# Autodesk Inventor assembly: base
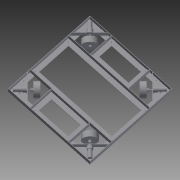
[picture p0: Inventor's stored thumbnail of the model, 180x180]
Saved by Autodesk Inventor 2015 (Build 190159000, 159)
## iProperties
Created: 2017-09-26
Part Number: base
Document SubType Name: Assembly
Designer: Anshul
Author: Anshul
## Documents named in this file (9)
- E:\robocon\throwing bot\base.iam
- E:\robocon\throwing bot\body_outer_L.ipt
- E:\robocon\throwing bot\body_inner_L_clamp.ipt
- E:\robocon\throwing bot\offcenter_L_clamp.ipt
- E:\robocon\throwing bot\offcentered_shaft_dc_and_encoder.ipt
- E:\robocon\throwing bot\omni_wheel.ipt
- E:\robocon\throwing bot\body_inner_center_bar.ipt
- E:\robocon\throwing bot\body_inner_L_support.ipt
- E:\robocon\throwing bot\body_inner_L_support(2).ipt
## Components (26 placed, 8 different names)
1. body_outer_L:1 — Mate:1, Flush:1, Mate:2, Flush:2, Mate:6, Mate:7, Mate:8, Mate:50, Mate:52
2. body_outer_L:2 — Mate:1, Flush:1, Mate:4, Mate:5, Mate:18, Mate:19, Mate:55, Mate:57, Mate:64, Mate:66
3. body_outer_L:3 — Mate:2, Flush:2, Mate:3, Flush:3, Mate:9, Mate:10, Mate:20, Mate:22, Mate:58, Mate:60, Mate:61, Mate:63
4. body_outer_L:4 — Mate:3, Mate:4, Flush:3, Mate:17, Mate:21, Mate:49, Mate:51, Mate:53, Mate:54
5. body_inner_L_clamp:1 — Mate:5, Mate:6, Mate:7, Mate:32, Mate:33, Mate:34
6. body_inner_L_clamp:2 — Mate:17, Mate:18, Mate:19, Mate:35, Mate:36, Mate:37
7. body_inner_L_clamp:3 — Mate:20, Mate:21, Mate:22, Mate:38, Mate:39, Mate:40
8. body_inner_L_clamp:4 — Mate:8, Mate:9, Mate:10, Mate:11, Mate:12, Mate:13
9. offcenter_L_clamp:1 — Mate:11, Mate:12, Mate:13, Mate:14, Mate:15, Mate:16
10. offcentered_shaft_dc_and_encoder:1 — Mate:14, Mate:15, Mate:16, Mate:45, Mate:48
11. offcenter_L_clamp:2 — Mate:35, Mate:36, Mate:37
12. offcentered_shaft_dc_and_encoder:2 — Mate:43, Mate:44
13. offcenter_L_clamp:3 — Mate:38, Mate:39, Mate:40
14. offcentered_shaft_dc_and_encoder:3 — Mate:46, Mate:47
15. offcenter_L_clamp:4 — Mate:32, Mate:33, Mate:34
16. offcentered_shaft_dc_and_encoder:4 — Mate:41, Mate:42
17. omni_wheel:1 — Mate:41, Mate:42
18. omni_wheel:2 — Mate:43, Mate:44
19. omni_wheel:3 — Mate:45, Mate:48
20. omni_wheel:4 — Mate:46, Mate:47
21. body_inner_center_bar:1 — Mate:49, Mate:50, Mate:54, Mate:59, Mate:62
22. body_inner_center_bar:2 — Mate:51, Mate:52, Mate:53, Mate:56, Mate:65
23. body_inner_L_support:1 — Mate:55, Mate:56, Mate:57
24. body_inner_L_support:2 — Mate:58, Mate:59, Mate:60
25. body_inner_L_support(2):1 — Mate:64, Mate:65, Mate:66
26. body_inner_L_support(2):2 — Mate:61, Mate:62, Mate:63
## Relationships (69: Mate 66, Flush 3)
- Mate:1: body_outer_L:1 ↔ body_outer_L:2
- Flush:1: body_outer_L:1 ↔ body_outer_L:2
- Mate:2: body_outer_L:1 ↔ body_outer_L:3
- Flush:2: body_outer_L:1 ↔ body_outer_L:3
- Mate:3: body_outer_L:3 ↔ body_outer_L:4
- Mate:4: body_outer_L:2 ↔ body_outer_L:4
- Flush:3: body_outer_L:3 ↔ body_outer_L:4
- Mate:5: body_outer_L:2 ↔ body_inner_L_clamp:1
- Mate:6: body_outer_L:1 ↔ body_inner_L_clamp:1
- Mate:7: body_outer_L:1 ↔ body_inner_L_clamp:1
- Mate:8: body_outer_L:1 ↔ body_inner_L_clamp:4
- Mate:9: body_outer_L:3 ↔ body_inner_L_clamp:4
- Mate:10: body_outer_L:3 ↔ body_inner_L_clamp:4
- Mate:11: body_inner_L_clamp:4 ↔ offcenter_L_clamp:1
- Mate:12: body_inner_L_clamp:4 ↔ offcenter_L_clamp:1
- Mate:13: body_inner_L_clamp:4 ↔ offcenter_L_clamp:1
- Mate:14: offcenter_L_clamp:1 ↔ offcentered_shaft_dc_and_encoder:1
- Mate:15: offcenter_L_clamp:1 ↔ offcentered_shaft_dc_and_encoder:1
- Mate:16: offcenter_L_clamp:1 ↔ offcentered_shaft_dc_and_encoder:1
- Mate:17: body_outer_L:4 ↔ body_inner_L_clamp:2
- Mate:18: body_outer_L:2 ↔ body_inner_L_clamp:2
- Mate:19: body_outer_L:2 ↔ body_inner_L_clamp:2
- Mate:20: body_outer_L:3 ↔ body_inner_L_clamp:3
- Mate:21: body_outer_L:4 ↔ body_inner_L_clamp:3
- Mate:22: body_outer_L:3 ↔ body_inner_L_clamp:3
- [Mate]: offcenter_L_clamp:2 ↔ offcentered_shaft_dc_and_encoder:2
- [Mate]: offcenter_L_clamp:2 ↔ offcentered_shaft_dc_and_encoder:2
- [Mate]: offcenter_L_clamp:2 ↔ offcentered_shaft_dc_and_encoder:2
- [Mate]: offcenter_L_clamp:3 ↔ offcentered_shaft_dc_and_encoder:3
- [Mate]: offcenter_L_clamp:3 ↔ offcentered_shaft_dc_and_encoder:3
- [Mate]: offcenter_L_clamp:3 ↔ offcentered_shaft_dc_and_encoder:3
- [Mate]: offcenter_L_clamp:4 ↔ offcentered_shaft_dc_and_encoder:4
- [Mate]: offcenter_L_clamp:4 ↔ offcentered_shaft_dc_and_encoder:4
- [Mate]: offcenter_L_clamp:4 ↔ offcentered_shaft_dc_and_encoder:4
- Mate:32: body_inner_L_clamp:1 ↔ offcenter_L_clamp:4
- Mate:33: body_inner_L_clamp:1 ↔ offcenter_L_clamp:4
- Mate:34: body_inner_L_clamp:1 ↔ offcenter_L_clamp:4
- Mate:35: body_inner_L_clamp:2 ↔ offcenter_L_clamp:2
- Mate:36: body_inner_L_clamp:2 ↔ offcenter_L_clamp:2
- Mate:37: body_inner_L_clamp:2 ↔ offcenter_L_clamp:2
- Mate:38: body_inner_L_clamp:3 ↔ offcenter_L_clamp:3
- Mate:39: body_inner_L_clamp:3 ↔ offcenter_L_clamp:3
- Mate:40: body_inner_L_clamp:3 ↔ offcenter_L_clamp:3
- Mate:41: offcentered_shaft_dc_and_encoder:4 ↔ omni_wheel:1
- Mate:42: offcentered_shaft_dc_and_encoder:4 ↔ omni_wheel:1
- Mate:43: offcentered_shaft_dc_and_encoder:2 ↔ omni_wheel:2
- Mate:44: offcentered_shaft_dc_and_encoder:2 ↔ omni_wheel:2
- Mate:45: offcentered_shaft_dc_and_encoder:1 ↔ omni_wheel:3
- Mate:46: offcentered_shaft_dc_and_encoder:3 ↔ omni_wheel:4
- Mate:47: offcentered_shaft_dc_and_encoder:3 ↔ omni_wheel:4
- Mate:48: offcentered_shaft_dc_and_encoder:1 ↔ omni_wheel:3
- Mate:49: body_outer_L:4 ↔ body_inner_center_bar:1
- Mate:50: body_outer_L:1 ↔ body_inner_center_bar:1
- Mate:51: body_outer_L:4 ↔ body_inner_center_bar:2
- Mate:52: body_outer_L:1 ↔ body_inner_center_bar:2
- Mate:53: body_outer_L:4 ↔ body_inner_center_bar:2
- Mate:54: body_outer_L:4 ↔ body_inner_center_bar:1
- Mate:55: body_outer_L:2 ↔ body_inner_L_support:1
- Mate:56: body_inner_center_bar:2 ↔ body_inner_L_support:1
- Mate:57: body_outer_L:2 ↔ body_inner_L_support:1
- Mate:58: body_outer_L:3 ↔ body_inner_L_support:2
- Mate:59: body_inner_center_bar:1 ↔ body_inner_L_support:2
- Mate:60: body_outer_L:3 ↔ body_inner_L_support:2
- Mate:61: body_outer_L:3 ↔ body_inner_L_support(2):2
- Mate:62: body_inner_center_bar:1 ↔ body_inner_L_support(2):2
- Mate:63: body_outer_L:3 ↔ body_inner_L_support(2):2
- Mate:64: body_outer_L:2 ↔ body_inner_L_support(2):1
- Mate:65: body_inner_center_bar:2 ↔ body_inner_L_support(2):1
- Mate:66: body_outer_L:2 ↔ body_inner_L_support(2):1
## Named parameters: d26_d17 = 0 mm, d27_d18 = 0 mm, d28_d19 = 0 mm, d29_d17 = 0 mm, d30_d18 = 0 mm, d31_d19 = 0 mm, d32_d17 = 0 mm, d33_d18 = 0 mm, d34_d19 = 0 mm
